# Autodesk Inventor assembly: Complete_robotic_arm
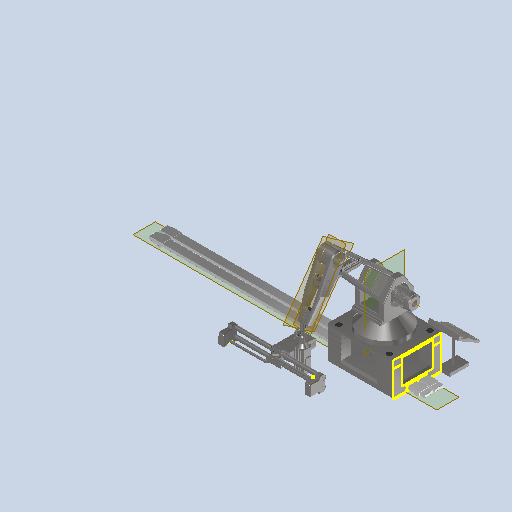
[picture p0: Inventor's stored thumbnail of the model, 512x512]
Saved by Autodesk Inventor 2023 (Build 270158000, 158)
## iProperties
Created: 2023-11-21
Part Number: Complete_robotic_arm
Document SubType Name: Assembly
Designer: Beatrice
Author: Beatrice
## Documents named in this file (7)
- E:\WORKSPACE_2\wheel_changing_assignment\Complete_robotic_arm.iam
- E:\WORKSPACE_2\wheel_changing_assignment\robotic_base_halfed.ipt
- E:\WORKSPACE_2\wheel_changing_assignment\robo_arm_base.ipt
- E:\WORKSPACE_2\wheel_changing_assignment\arm_assembly.iam
- E:\WORKSPACE_2\wheel_changing_assignment\slider.ipt
- E:\WORKSPACE_2\wheel_changing_assignment\reduced_ctrl_panel.ipt
- E:\WORKSPACE_2\wheel_changing_assignment\driver_motor.ipt
## Components (6 placed, 6 different names)
1. robotic_base_halfed:1 — Mate:1, Mate:2, Mate:3, Flush:2, Flush:3, Mate:5, Flush:4, Mate:6, Flush:5
2. robo_arm_base:1 — Mate:1, Mate:2, Mate:3, Mate:4, Flush:1, Angle:1, Mate:7, Flush:6
3. arm_assembly:1 [sub-assembly] — Mate:4, Flush:1, Angle:1
4. slider:1 — Flush:2, Flush:3, Mate:5
5. reduced_ctrl_panel:1 — Flush:4, Mate:6, Flush:5
6. driver_motor:1 — Mate:7, Flush:6
## Relationships (14: Mate 7, Flush 6, Angle 1)
- Mate:1: robotic_base_halfed:1 ↔ robo_arm_base:1
- Mate:2: robotic_base_halfed:1 ↔ robo_arm_base:1
- Mate:3: robotic_base_halfed:1 ↔ robo_arm_base:1
- Mate:4: robo_arm_base:1 ↔ arm_assembly:1
- Flush:1: robo_arm_base:1 ↔ arm_assembly:1
- Angle:1 (-45 deg): robo_arm_base:1 ↔ arm_assembly:1
- Flush:2: robotic_base_halfed:1 ↔ slider:1
- Flush:3: robotic_base_halfed:1 ↔ slider:1
- Mate:5 (2 mm): robotic_base_halfed:1 ↔ slider:1
- Flush:4: robotic_base_halfed:1 ↔ reduced_ctrl_panel:1
- Mate:6: robotic_base_halfed:1 ↔ reduced_ctrl_panel:1
- Flush:5 (5 mm): robotic_base_halfed:1 ↔ reduced_ctrl_panel:1
- Mate:7: robo_arm_base:1 ↔ driver_motor:1
- Flush:6 (4 mm): robo_arm_base:1 ↔ driver_motor:1
